# Autodesk Inventor assembly: Z Axis
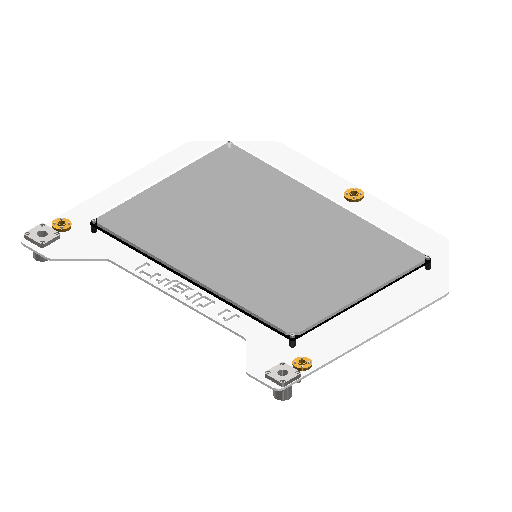
[picture p0: Inventor's stored thumbnail of the model, 512x512]
Saved by Autodesk Inventor 2023.2 (Build 272271000, 271)
## iProperties
Created: 2023-02-02
Part Number: Z Axis
Document SubType Name: Assembly
Designer: remop
Author: remop
## Documents named in this file (10)
- C:\Users\remop\OneDrive\Documents\Inventor\3D Printers\LuEVO\Mk5_FullKinematic\Z Axis.iam
- C:\Users\remop\OneDrive\Documents\Inventor\3D Printers\LuEVO\Mk5_FullKinematic\Z Axis Base.ipt
- C:\Users\remop\OneDrive\Documents\Inventor\3D Printers\LuEVO\Mk5_FullKinematic\E3D High Temperature Bed 300x200.ipt
- C:\Users\remop\OneDrive\Documents\Inventor\3D Printers\LuEVO\Mk5_FullKinematic\Z Axis Bearing.ipt
- C:\Users\remop\OneDrive\Documents\Inventor\3D Printers\LuEVO\Mk5_FullKinematic\Z Axis Nut.ipt
- C:\Users\remop\OneDrive\Documents\Inventor\3D Printers\LuEVO\Mk5_FullKinematic\Heated Bed Spacer.ipt
- C:\Users\remop\OneDrive\Documents\Inventor\3D Printers\LuEVO\Mk5_FullKinematic\Heated Bed Glass.ipt
- C:\Users\remop\OneDrive\Documents\Inventor\Content Center Files\R2023\en-US\AS 1420\AS 1420 - 1973 - M3 x 10.ipt
- C:\Users\remop\OneDrive\Documents\Inventor\Content Center Files\R2023\en-US\AS 1420\AS 1420 - 1973 - M3 x 8.ipt
- C:\Users\remop\OneDrive\Documents\Inventor\Content Center Files\R2023\en-US\AS 1112 (2)\AS 1112 - M4  Type 5.ipt
## Components (48 placed, 9 different names)
1. Z Axis Base:1 — Rotational:1, Cylindrical:1, Rigid:6, Rigid:7, Rigid:8, Rigid:9, Insert:9, Insert:10, Insert:11, Insert:12, Rigid:10, Rigid:11, Rigid:12, Rigid:13, Rigid:14, Insert:13, Insert:14, Insert:15, Insert:16, Insert:17, Insert:18, Insert:19, Insert:20, Insert:21, Insert:22, Insert:23, Insert:24, Insert:33, Insert:34, Insert:35, Insert:36, Insert:37, Insert:38, Insert:39, Insert:40
2. E3D High Temperature Bed 300x200:1 — Rotational:1, Cylindrical:1, Flush:1, Flush:2, Flush:3, Insert:1, Insert:4, Insert:6, Insert:8
3. Z Axis Bearing:1 — Rigid:12, Insert:25, Insert:26, Insert:27, Insert:28
4. Z Axis Bearing:2 — Rigid:11, Insert:29, Insert:30, Insert:31, Insert:32
5. Z Axis Nut:1 — Rigid:10
6. Z Axis Nut:2 — Rigid:13
7. Z Axis Nut:3 — Rigid:14
8. Heated Bed Spacer:2 — Rigid:7
9. Heated Bed Spacer:3 — Rigid:8
10. Heated Bed Spacer:4 — Rigid:9
11. Heated Bed Spacer:5 — Rigid:6
12. Heated Bed Glass:1 — Flush:1, Flush:2, Flush:3
13. AS 1420 - Metric M3 x 10:1 — Insert:1
14. AS 1420 - Metric M3 x 10:4 — Insert:4
15. AS 1420 - Metric M3 x 10:6 — Insert:6
16. AS 1420 - Metric M3 x 10:8 — Insert:8
17. AS 1420 - Metric M3 x 10:9 — Insert:9
18. AS 1420 - Metric M3 x 10:10 — Insert:10
19. AS 1420 - Metric M3 x 10:11 — Insert:11
20. AS 1420 - Metric M3 x 10:12 — Insert:12
21. AS 1420 - Metric M3 x 8:1 — Insert:13
22. AS 1420 - Metric M3 x 8:2 — Insert:14
23. AS 1420 - Metric M3 x 8:3 — Insert:15
24. AS 1420 - Metric M3 x 8:4 — Insert:16
25. AS 1420 - Metric M3 x 8:5 — Insert:17
26. AS 1420 - Metric M3 x 8:6 — Insert:18
27. AS 1420 - Metric M3 x 8:7 — Insert:19
28. AS 1420 - Metric M3 x 8:8 — Insert:20
29. AS 1420 - Metric M3 x 8:9 — Insert:21
30. AS 1420 - Metric M3 x 8:10 — Insert:22
31. AS 1420 - Metric M3 x 8:11 — Insert:23
32. AS 1420 - Metric M3 x 8:12 — Insert:24
33. AS 1420 - Metric M3 x 8:13 — Insert:25
34. AS 1420 - Metric M3 x 8:14 — Insert:26
35. AS 1420 - Metric M3 x 8:15 — Insert:27
36. AS 1420 - Metric M3 x 8:16 — Insert:28
37. AS 1420 - Metric M3 x 8:17 — Insert:29
38. AS 1420 - Metric M3 x 8:18 — Insert:30
39. AS 1420 - Metric M3 x 8:19 — Insert:31
40. AS 1420 - Metric M3 x 8:20 — Insert:32
41. AS 1112 (2) - Metric M4  Type 5:1 — Insert:33
42. AS 1112 (2) - Metric M4  Type 5:2 — Insert:34
43. AS 1112 (2) - Metric M4  Type 5:3 — Insert:35
44. AS 1112 (2) - Metric M4  Type 5:4 — Insert:36
45. AS 1112 (2) - Metric M4  Type 5:5 — Insert:37
46. AS 1112 (2) - Metric M4  Type 5:6 — Insert:38
47. AS 1112 (2) - Metric M4  Type 5:7 — Insert:39
48. AS 1112 (2) - Metric M4  Type 5:8 — Insert:40
## Relationships (50: Insert 36, WeldJoint 9, Flush 3, RevoluteJoint 1, CylindricalJoint 1)
- Rotational:1 [RevoluteJoint] (10 mm): Z Axis Base:1 ↔ E3D High Temperature Bed 300x200:1
- Cylindrical:1: Z Axis Base:1 ↔ E3D High Temperature Bed 300x200:1
- Rigid:6 [WeldJoint]: Z Axis Base:1 ↔ Heated Bed Spacer:5
- Rigid:7 [WeldJoint]: Z Axis Base:1 ↔ Heated Bed Spacer:2
- Rigid:8 [WeldJoint]: Z Axis Base:1 ↔ Heated Bed Spacer:3
- Rigid:9 [WeldJoint]: Z Axis Base:1 ↔ Heated Bed Spacer:4
- Flush:1: E3D High Temperature Bed 300x200:1 ↔ Heated Bed Glass:1
- Flush:2: E3D High Temperature Bed 300x200:1 ↔ Heated Bed Glass:1
- Flush:3 (1 mm): E3D High Temperature Bed 300x200:1 ↔ Heated Bed Glass:1
- Insert:1: E3D High Temperature Bed 300x200:1 ↔ AS 1420 - Metric M3 x 10:1
- Insert:4: E3D High Temperature Bed 300x200:1 ↔ AS 1420 - Metric M3 x 10:4
- Insert:6: E3D High Temperature Bed 300x200:1 ↔ AS 1420 - Metric M3 x 10:6
- Insert:8: E3D High Temperature Bed 300x200:1 ↔ AS 1420 - Metric M3 x 10:8
- Insert:9: Z Axis Base:1 ↔ AS 1420 - Metric M3 x 10:9
- Insert:10: Z Axis Base:1 ↔ AS 1420 - Metric M3 x 10:10
- Insert:11: Z Axis Base:1 ↔ AS 1420 - Metric M3 x 10:11
- Insert:12: Z Axis Base:1 ↔ AS 1420 - Metric M3 x 10:12
- Rigid:10 [WeldJoint]: Z Axis Base:1 ↔ Z Axis Nut:1
- Rigid:11 [WeldJoint]: Z Axis Base:1 ↔ Z Axis Bearing:2
- Rigid:12 [WeldJoint]: Z Axis Base:1 ↔ Z Axis Bearing:1
- Rigid:13 [WeldJoint]: Z Axis Base:1 ↔ Z Axis Nut:2
- Rigid:14 [WeldJoint]: Z Axis Base:1 ↔ Z Axis Nut:3
- Insert:13: Z Axis Base:1 ↔ AS 1420 - Metric M3 x 8:1
- Insert:14: Z Axis Base:1 ↔ AS 1420 - Metric M3 x 8:2
- Insert:15: Z Axis Base:1 ↔ AS 1420 - Metric M3 x 8:3
- Insert:16: Z Axis Base:1 ↔ AS 1420 - Metric M3 x 8:4
- Insert:17: Z Axis Base:1 ↔ AS 1420 - Metric M3 x 8:5
- Insert:18: Z Axis Base:1 ↔ AS 1420 - Metric M3 x 8:6
- Insert:19: Z Axis Base:1 ↔ AS 1420 - Metric M3 x 8:7
- Insert:20: Z Axis Base:1 ↔ AS 1420 - Metric M3 x 8:8
- Insert:21: Z Axis Base:1 ↔ AS 1420 - Metric M3 x 8:9
- Insert:22: Z Axis Base:1 ↔ AS 1420 - Metric M3 x 8:10
- Insert:23: Z Axis Base:1 ↔ AS 1420 - Metric M3 x 8:11
- Insert:24: Z Axis Base:1 ↔ AS 1420 - Metric M3 x 8:12
- Insert:25: Z Axis Bearing:1 ↔ AS 1420 - Metric M3 x 8:13
- Insert:26: Z Axis Bearing:1 ↔ AS 1420 - Metric M3 x 8:14
- Insert:27: Z Axis Bearing:1 ↔ AS 1420 - Metric M3 x 8:15
- Insert:28: Z Axis Bearing:1 ↔ AS 1420 - Metric M3 x 8:16
- Insert:29: Z Axis Bearing:2 ↔ AS 1420 - Metric M3 x 8:17
- Insert:30: Z Axis Bearing:2 ↔ AS 1420 - Metric M3 x 8:18
- Insert:31: Z Axis Bearing:2 ↔ AS 1420 - Metric M3 x 8:19
- Insert:32: Z Axis Bearing:2 ↔ AS 1420 - Metric M3 x 8:20
- Insert:33: Z Axis Base:1 ↔ AS 1112 (2) - Metric M4  Type 5:1
- Insert:34: Z Axis Base:1 ↔ AS 1112 (2) - Metric M4  Type 5:2
- Insert:35: Z Axis Base:1 ↔ AS 1112 (2) - Metric M4  Type 5:3
- Insert:36: Z Axis Base:1 ↔ AS 1112 (2) - Metric M4  Type 5:4
- Insert:37: Z Axis Base:1 ↔ AS 1112 (2) - Metric M4  Type 5:5
- Insert:38: Z Axis Base:1 ↔ AS 1112 (2) - Metric M4  Type 5:6
- Insert:39: Z Axis Base:1 ↔ AS 1112 (2) - Metric M4  Type 5:7
- Insert:40: Z Axis Base:1 ↔ AS 1112 (2) - Metric M4  Type 5:8
